# Autodesk Inventor assembly: loader
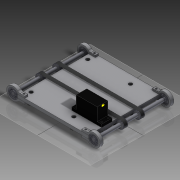
[picture p0: Inventor's stored thumbnail of the model, 180x180]
Saved by Autodesk Inventor 2013 (Build 170138000, 138)
## iProperties
Created: 2013-09-15
Part Number: loader
Document SubType Name: Assembly
Designer: Ian
Mass: 307.738 g
Surface Area: 897.592 cm^2
Volume: 183.399 cm^3
Density: 1.67797 g/cm^3
Author: Ian
## Documents named in this file (8)
- C:\Users\Ian\Documents\Inventor\xyPartStorage\loader\loader.iam
- C:\Users\Ian\Documents\Inventor\xyPartStorage\loader\loader_frame.ipt
- C:\Users\Ian\Documents\Inventor\xyPartStorage\loader\bearing_blcok.ipt
- C:\Users\Ian\Documents\Inventor\Content Center Files\R2013\en-US\ANSI SKF EEB(2)\SKFEEB 2-ZANSI.ipt
- C:\Users\Ian\Documents\Inventor\xyPartStorage\loader\loader\Design Accelerator\Shaft1.iam
- C:\Users\Ian\Documents\Inventor\xyPartStorage\loader\loader\Design Accelerator\Synchronous Belts Transmission1.iam
- C:\Users\Ian\Documents\Inventor\xyPartStorage\loader\servo.iam
- C:\Users\Ian\Documents\Inventor\xyPartStorage\loader\1_5 inch spacer.ipt
## Components (18 placed, 7 different names)
1. loader_frame:1 — Mate:1, Mate:2, Mate:3, Mate:4, Tangent:1, Flush:2, Tangent:2, Flush:3, Tangent:3, Flush:5, Flush:6, Tangent:4, Angle:1, Mate:17, Flush:8, Flush:9, Mate:18, Mate:19, Mate:20, Mate:21, Mate:22, Mate:23, Mate:24, Mate:25
2. bearing_blcok:1 — Mate:1, Mate:6, Flush:6, Flush:7
3. bearing_blcok:2 — Mate:2, Mate:5, Flush:4, Flush:5, Mate:16
4. bearing_blcok:3 — Mate:4, Flush:1, Insert:1, Flush:2, Mate:14
5. bearing_blcok:4 — Mate:3, Insert:2, Flush:3, Mate:8, Mate:11
6. SKF Series EEB - Type Z EEB 2-Z:1 — Flush:1, Tangent:1, Insert:1
7. SKF Series EEB - Type Z EEB 2-Z:2 — Mate:6, Flush:7, Tangent:4, Mate:15
8. SKF Series EEB - Type Z EEB 2-Z:3 — Mate:5, Flush:4, Tangent:3, Mate:10
9. SKF Series EEB - Type Z EEB 2-Z:4 — Insert:2, Tangent:2, Mate:7
10. Shaft:1 [sub-assembly] — Mate:7, Mate:8, Angle:1, Mate:9
11. Synchronous Belts Transmission:1 [sub-assembly] — Mate:9, Mate:10, Mate:11, Mate:12, Mate:13
12. Synchronous Belts Transmission:2 [sub-assembly] — Mate:12, Mate:13, Mate:14
13. Shaft:2 [sub-assembly] — Mate:15, Mate:16
14. servo:1 [sub-assembly] — Mate:17, Flush:8, Flush:9
15. 1_5 inch spacer:1 — Mate:22, Mate:23
16. 1_5 inch spacer:2 — Mate:20, Mate:21
17. 1_5 inch spacer:3 — Mate:24, Mate:25
18. 1_5 inch spacer:4 — Mate:18, Mate:19
## Relationships (41: Mate 25, Flush 9, Tangent 4, Insert 2, Angle 1)
- Mate:1: loader_frame:1 ↔ bearing_blcok:1
- Mate:2: loader_frame:1 ↔ bearing_blcok:2
- Mate:3: loader_frame:1 ↔ bearing_blcok:4
- Mate:4: loader_frame:1 ↔ bearing_blcok:3
- Flush:1: bearing_blcok:3 ↔ SKF Series EEB - Type Z EEB 2-Z:1
- Tangent:1: loader_frame:1 ↔ SKF Series EEB - Type Z EEB 2-Z:1
- Insert:1: bearing_blcok:3 ↔ SKF Series EEB - Type Z EEB 2-Z:1
- Flush:2: loader_frame:1 ↔ bearing_blcok:3
- Insert:2: bearing_blcok:4 ↔ SKF Series EEB - Type Z EEB 2-Z:4
- Tangent:2: loader_frame:1 ↔ SKF Series EEB - Type Z EEB 2-Z:4
- Flush:3: loader_frame:1 ↔ bearing_blcok:4
- Mate:5: bearing_blcok:2 ↔ SKF Series EEB - Type Z EEB 2-Z:3
- Flush:4: bearing_blcok:2 ↔ SKF Series EEB - Type Z EEB 2-Z:3
- Tangent:3: loader_frame:1 ↔ SKF Series EEB - Type Z EEB 2-Z:3
- Flush:5: loader_frame:1 ↔ bearing_blcok:2
- Mate:6: bearing_blcok:1 ↔ SKF Series EEB - Type Z EEB 2-Z:2
- Flush:6: loader_frame:1 ↔ bearing_blcok:1
- Flush:7: bearing_blcok:1 ↔ SKF Series EEB - Type Z EEB 2-Z:2
- Tangent:4: loader_frame:1 ↔ SKF Series EEB - Type Z EEB 2-Z:2
- Mate:7: SKF Series EEB - Type Z EEB 2-Z:4 ↔ Shaft:1
- Mate:8: bearing_blcok:4 ↔ Shaft:1
- Angle:1 (0 deg): loader_frame:1 ↔ Shaft:1
- Mate:9: Shaft:1 ↔ Synchronous Belts Transmission:1
- Mate:10: SKF Series EEB - Type Z EEB 2-Z:3 ↔ Synchronous Belts Transmission:1
- Mate:11 (44.45 mm): bearing_blcok:4 ↔ Synchronous Belts Transmission:1
- Mate:12: Synchronous Belts Transmission:1 ↔ Synchronous Belts Transmission:2
- Mate:13: Synchronous Belts Transmission:1 ↔ Synchronous Belts Transmission:2
- Mate:14 (44.45 mm): bearing_blcok:3 ↔ Synchronous Belts Transmission:2
- Mate:15: SKF Series EEB - Type Z EEB 2-Z:2 ↔ Shaft:2
- Mate:16: bearing_blcok:2 ↔ Shaft:2
- Mate:17: loader_frame:1 ↔ servo:1
- Flush:8 (25.4 mm): loader_frame:1 ↔ servo:1
- Flush:9: loader_frame:1 ↔ servo:1
- Mate:18: loader_frame:1 ↔ 1_5 inch spacer:4
- Mate:19: loader_frame:1 ↔ 1_5 inch spacer:4
- Mate:20: loader_frame:1 ↔ 1_5 inch spacer:2
- Mate:21: loader_frame:1 ↔ 1_5 inch spacer:2
- Mate:22: loader_frame:1 ↔ 1_5 inch spacer:1
- Mate:23: loader_frame:1 ↔ 1_5 inch spacer:1
- Mate:24: loader_frame:1 ↔ 1_5 inch spacer:3
- Mate:25: loader_frame:1 ↔ 1_5 inch spacer:3
